# Autodesk Inventor assembly: 6P Sprocket
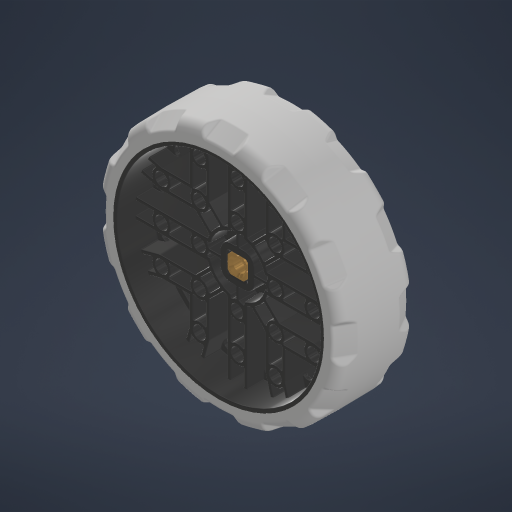
[picture p0: Inventor's stored thumbnail of the model, 512x512]
Saved by Autodesk Inventor 2024 (Build 280153000, 153)
## iProperties
Created: 2022-08-02
Part Number: 6P Sprocket
Document SubType Name: Assembly
Designer: ylu12
Author: ylu12
## Documents named in this file (4)
- \\Mac\Home\Desktop\code\1599V-VRC\Cad\Motion\Wheels\Traction Wheel\3.25 Traction AS, Circle.iam
- \\Mac\Home\Desktop\code\1599V-VRC\Cad\Motion\Wheels\Reference Files\3.25 Traction Antistatic.ipt
- \\Mac\Home\Desktop\code\1599V-VRC\Cad\Motion\HS Shaft Adapter Circle.ipt
- \\Mac\Home\Desktop\code\1599V-VRC\Cad\Motion\Wheels\Traction Wheel.iam
## Components (2 placed, 2 different names)
1. 3.25 Traction Antistatic:1 — Mate:20, Mate:22, Mate:24
2. Circle — Mate:32, Mate:33, Flush:10
## Relationships (6: Mate 5, Flush 1)
- Mate:20: 3.25 Traction Antistatic:1
- Mate:22: 3.25 Traction Antistatic:1
- Mate:24: 3.25 Traction Antistatic:1
- Mate:32: Circle
- Mate:33: Circle
- Flush:10 (6.35 mm): Circle
## Named parameters: Thickness = 8.255 mm
